# Autodesk Inventor assembly: Leg
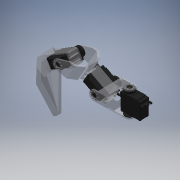
[picture p0: Inventor's stored thumbnail of the model, 180x180]
Saved by Autodesk Inventor 2016 (Build 200138000, 138)
## iProperties
Created: 2016-05-19
Part Number: Leg
Document SubType Name: Assembly
Designer: kromm.je.s
Author: kromm.je.s
## Documents named in this file (5)
- H:\CAD\Hexapod\Leg.iam
- H:\CAD\Hexapod\turnigy-tgy-s901d-digital-servo-1.snapshot.5 (1)\S901D.iam
- H:\CAD\Hexapod\Servo Bracket.ipt
- H:\CAD\Hexapod\Servo Bracket 2.ipt
- H:\CAD\Hexapod\Servo Bracket 3.ipt
## Components (6 placed, 4 different names)
1. S901D:1 [sub-assembly] — Mate:2, Mate:4, Mate:5, Mate:6, Mate:7, Mate:8
2. S901D:2 [sub-assembly] — Mate:1, Mate:3, Angle:1
3. Servo Bracket:1 — Mate:1, Mate:2, Mate:3, Mate:4, Mate:5, Angle:1, Angle:2
4. Servo Bracket 2:1 — Mate:6, Mate:7, Mate:8, Mate:9, Mate:10, Angle:2, Angle:3
5. S901D:3 [sub-assembly] — Mate:9, Mate:10, Mate:11, Mate:12, Mate:13
6. Servo Bracket 3:1 — Mate:11, Mate:12, Mate:13, Angle:3
## Relationships (16: Mate 13, Angle 3)
- Mate:1: S901D:2 ↔ Servo Bracket:1
- Mate:2: S901D:1 ↔ Servo Bracket:1
- Mate:3: S901D:2 ↔ Servo Bracket:1
- Mate:4: S901D:1 ↔ Servo Bracket:1
- Mate:5: S901D:1 ↔ Servo Bracket:1
- Mate:6: S901D:1 ↔ Servo Bracket 2:1
- Mate:7: S901D:1 ↔ Servo Bracket 2:1
- Mate:8: S901D:1 ↔ Servo Bracket 2:1
- Mate:9: Servo Bracket 2:1 ↔ S901D:3
- Mate:10: Servo Bracket 2:1 ↔ S901D:3
- Angle:1 (0 deg): S901D:2 ↔ Servo Bracket:1
- Mate:11: S901D:3 ↔ Servo Bracket 3:1
- Mate:12: S901D:3 ↔ Servo Bracket 3:1
- Mate:13: S901D:3 ↔ Servo Bracket 3:1
- Angle:2 (-30 deg): Servo Bracket:1 ↔ Servo Bracket 2:1
- Angle:3 (60 deg): Servo Bracket 2:1 ↔ Servo Bracket 3:1
